# Autodesk Inventor assembly: Sounder
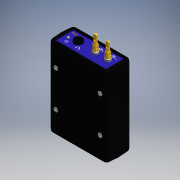
[picture p0: Inventor's stored thumbnail of the model, 180x180]
Saved by Autodesk Inventor 2016 (Build 200138000, 138)
## iProperties
Created: 2016-12-24
Part Number: Sounder
Document SubType Name: Assembly
Designer: Tyler
Author: Tyler
## Documents named in this file (11)
- C:\Users\Tyler\Documents\Small Projects\Personal\morse-practice-oscillator\Mechanicial\Sounder\Sounder.iam
- C:\Users\Tyler\Documents\Small Projects\Personal\morse-practice-oscillator\Mechanicial\Sounder\Imported Components\1593L BOTTOM\1593L BOTTOM.ipt
- C:\Users\Tyler\Documents\Small Projects\Personal\morse-practice-oscillator\Mechanicial\Sounder\PCB.iam
- C:\Users\Tyler\Documents\Small Projects\Personal\morse-practice-oscillator\Mechanicial\Sounder\Imported Components\1593L Top\1593L Top.ipt
- C:\Users\Tyler\Documents\Inventor\Content Center Files\R2016\en-US\ANSI B18.6.4(00)\ANSI B18.6.4 - 4-24 - 0.875(41) AB II.ipt
- C:\Users\Tyler\Documents\Small Projects\Personal\morse-practice-oscillator\Mechanicial\Sounder\frontPlate.ipt
- C:\Users\Tyler\Documents\Small Projects\Personal\morse-practice-oscillator\Mechanicial\Sounder\rearPlate_PP.ipt
- C:\Users\Tyler\Documents\Inventor\Content Center Files\R2016\en-US\BS 4183(1)\BS 4183 - M6(1).ipt
- C:\Users\Tyler\Documents\Small Projects\Personal\morse-practice-oscillator\Mechanicial\Sounder\rearPlate_jack.ipt
- C:\Users\Tyler\Documents\Small Projects\Personal\morse-practice-oscillator\Mechanicial\Sounder\dial rear.ipt
- C:\Users\Tyler\Documents\Small Projects\Personal\morse-practice-oscillator\Mechanicial\Sounder\dial front.ipt
## Components (15 placed, 10 different names)
1. 1593L BOTTOM:1 — Insert:1, Insert:2, Mate:5, Mate:6, Flush:1, Flush:8, Mate:8, Mate:9, Mate:10, Mate:11, Mate:12, Flush:9, Flush:10, Flush:11, Flush:12, Mate:13, Mate:14, Mate:15, Mate:18, Mate:19, Mate:20, Mate:23, Mate:25, Mate:26
2. PCB:1 [sub-assembly] — Insert:1, Insert:2, Mate:21, Mate:27, Mate:28, Mate:29, Mate:30, Mate:31, Mate:32, Mate:33, Mate:34, Mate:35, Mate:36
3. frontPlate:1 — Mate:13, Mate:14, Mate:15, Mate:22
4. rearPlate_PP:1 — Mate:18, Mate:19, Mate:20
5. 1593L Top:1 — Mate:5, Mate:6
6. Cross Recessed Flat Countersunk Head Tapping Screw - Type AB - Type II - Inch No. 4 - 24 -  7/8:1 — Mate:9, Flush:12
7. Cross Recessed Flat Countersunk Head Tapping Screw - Type AB - Type II - Inch No. 4 - 24 -  7/8:2 — Mate:10, Flush:11
8. Cross Recessed Flat Countersunk Head Tapping Screw - Type AB - Type II - Inch No. 4 - 24 -  7/8:3 — Mate:11, Flush:9
9. Cross Recessed Flat Countersunk Head Tapping Screw - Type AB - Type II - Inch No. 4 - 24 -  7/8:4 — Mate:12, Flush:10
10. BS 4183 - Metric M6:1 — Mate:21, Mate:22
11. rearPlate_jack:1 — Mate:23, Mate:25, Mate:26
12. dial rear:1 — Mate:27, Mate:29
13. dial rear:2 — Mate:28, Mate:30
14. dial front:1 — Mate:31, Mate:32, Mate:33
15. dial front:2 — Mate:34, Mate:35, Mate:36
## Relationships (36: Mate 28, Flush 6, Insert 2)
- Insert:1: 1593L BOTTOM:1 ↔ PCB:1
- Insert:2: 1593L BOTTOM:1 ↔ PCB:1
- Mate:5: 1593L BOTTOM:1 ↔ 1593L Top:1
- Mate:6: 1593L BOTTOM:1 ↔ 1593L Top:1
- Flush:1: 1593L BOTTOM:1
- Flush:8: 1593L BOTTOM:1
- Mate:8: 1593L BOTTOM:1
- Mate:9: 1593L BOTTOM:1 ↔ Cross Recessed Flat Countersunk Head Tapping Screw - Type AB - Type II - Inch No. 4 - 24 -  7/8:1
- Mate:10: 1593L BOTTOM:1 ↔ Cross Recessed Flat Countersunk Head Tapping Screw - Type AB - Type II - Inch No. 4 - 24 -  7/8:2
- Mate:11: 1593L BOTTOM:1 ↔ Cross Recessed Flat Countersunk Head Tapping Screw - Type AB - Type II - Inch No. 4 - 24 -  7/8:3
- Mate:12: 1593L BOTTOM:1 ↔ Cross Recessed Flat Countersunk Head Tapping Screw - Type AB - Type II - Inch No. 4 - 24 -  7/8:4
- Flush:9: 1593L BOTTOM:1 ↔ Cross Recessed Flat Countersunk Head Tapping Screw - Type AB - Type II - Inch No. 4 - 24 -  7/8:3
- Flush:10: 1593L BOTTOM:1 ↔ Cross Recessed Flat Countersunk Head Tapping Screw - Type AB - Type II - Inch No. 4 - 24 -  7/8:4
- Flush:11: 1593L BOTTOM:1 ↔ Cross Recessed Flat Countersunk Head Tapping Screw - Type AB - Type II - Inch No. 4 - 24 -  7/8:2
- Flush:12: 1593L BOTTOM:1 ↔ Cross Recessed Flat Countersunk Head Tapping Screw - Type AB - Type II - Inch No. 4 - 24 -  7/8:1
- Mate:13: 1593L BOTTOM:1 ↔ frontPlate:1
- Mate:14 (0.4 mm): 1593L BOTTOM:1 ↔ frontPlate:1
- Mate:15 (0.2 mm): 1593L BOTTOM:1 ↔ frontPlate:1
- Mate:18 (0.4 mm): 1593L BOTTOM:1 ↔ rearPlate_PP:1
- Mate:19: 1593L BOTTOM:1 ↔ rearPlate_PP:1
- Mate:20 (0.2 mm): 1593L BOTTOM:1 ↔ rearPlate_PP:1
- Mate:21: PCB:1 ↔ BS 4183 - Metric M6:1
- Mate:22: frontPlate:1 ↔ BS 4183 - Metric M6:1
- Mate:23: 1593L BOTTOM:1 ↔ rearPlate_jack:1
- Mate:25 (0.2 mm): 1593L BOTTOM:1 ↔ rearPlate_jack:1
- Mate:26 (0.4 mm): 1593L BOTTOM:1 ↔ rearPlate_jack:1
- Mate:27: PCB:1 ↔ dial rear:1
- Mate:28: PCB:1 ↔ dial rear:2
- Mate:29: PCB:1 ↔ dial rear:1
- Mate:30: PCB:1 ↔ dial rear:2
- Mate:31: PCB:1 ↔ dial front:1
- Mate:32: PCB:1 ↔ dial front:1
- Mate:33: PCB:1 ↔ dial front:1
- Mate:34: PCB:1 ↔ dial front:2
- Mate:35: PCB:1 ↔ dial front:2
- Mate:36: PCB:1 ↔ dial front:2
